# Autodesk Inventor assembly: coupler extention arm collector bottom
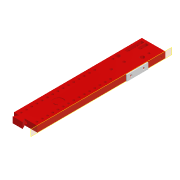
[picture p0: Inventor's stored thumbnail of the model, 180x180]
Saved by Autodesk Inventor 2020 (Build 240168000, 168)
## iProperties
Created: 2019-12-31
Part Number: coupler extention arm collector bottom
Document SubType Name: Assembly
Designer: ball
Author: ball
## Documents named in this file (3)
- C:\FTC\FTC8863CAD\2019 Robot\Delivery\extension arm\coupler extention arm collector bottom.iam
- C:\FTC\FTC8863CAD\2019 Robot\Delivery\extension arm\Coupler extension arm short edited holes for servo.ipt
- C:\FTC\FTC8863CAD\2019 Robot\Delivery\extension arm\standoff for gripper servo.ipt
## Components (2 placed, 2 different names)
1. Coupler extension arm short edited holes for servo:1 — Flush:1, Flush:2
2. standoff for gripper servo:1 — Flush:1, Flush:2
## Relationships (2: Flush 2)
- Flush:1: Coupler extension arm short edited holes for servo:1 ↔ standoff for gripper servo:1
- Flush:2: Coupler extension arm short edited holes for servo:1 ↔ standoff for gripper servo:1
